# Autodesk Inventor assembly: Gimbal Assembly
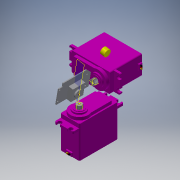
[picture p0: Inventor's stored thumbnail of the model, 180x180]
Saved by Autodesk Inventor 2016 (Build 200138000, 138)
## iProperties
Created: 2016-02-11
Part Number: Gimbal Assembly
Document SubType Name: Assembly
Designer: RoksBot
Author: RoksBot
## Documents named in this file (4)
- C:\Users\RoksBot\Documents\Inventor\Camera Mount\Gimbal Assembly.iam
- C:\Users\RoksBot\Documents\Inventor\Camera Mount\Servo Horn.ipt
- C:\Users\RoksBot\Documents\Inventor\Camera Mount\servo.ipt
- C:\Users\RoksBot\Documents\Inventor\Camera Mount\Camera.ipt
## Components (5 placed, 3 different names)
1. Servo Horn:1 — Insert:2, Mate:3
2. servo:1 — Insert:1, Mate:1, Pan Left-Right
3. Servo Horn:2 — Insert:1, Flush:1, Mate:2, Flush:2
4. servo:2 — Insert:2, Mate:1, Flush:1, Mate:2, Pan Left-Right
5. Camera:1 — Mate:3, Flush:2
## Relationships (8: Mate 3, Insert 2, Flush 2, Angle 1)
- Insert:1: servo:1 ↔ Servo Horn:2
- Insert:2: Servo Horn:1 ↔ servo:2
- Mate:1 (7.62 mm): servo:1 ↔ servo:2
- Flush:1 (-9.7282 mm): Servo Horn:2 ↔ servo:2
- Mate:2 (19.05 mm): Servo Horn:2 ↔ servo:2
- Pan Left-Right [Angle] (0 deg): servo:1 ↔ servo:2
- Mate:3: Servo Horn:1 ↔ Camera:1
- Flush:2: Servo Horn:2 ↔ Camera:1
